# Autodesk Inventor assembly: ForearmActuatorBody
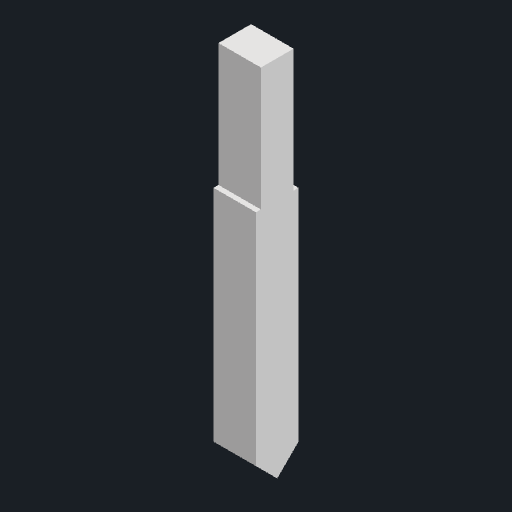
[picture p0: Inventor's stored thumbnail of the model, 512x512]
Saved by Autodesk Inventor 2023 (Build 270158000, 158)
## iProperties
Created: 2023-03-25
Part Number: ForearmActuatorBody
Document SubType Name: Assembly
Designer: Val
Author: Val
## Documents named in this file (3)
- C:\Users\valer\Desktop\str1ker\cad\external\ForearmActuator\ForearmActuatorBody.iam
- C:\Users\valer\Desktop\str1ker\cad\external\ForearmActuator\ForearmActuatorBody.ipt
- C:\Users\valer\Desktop\str1ker\cad\external\ForearmActuator\ForearmActuatorBodyBoundingBoxReal.ipt
## Components (2 placed, 2 different names)
1. ForearmActuatorBody:1 — Angle:1, Angle:2, Mate:1
2. ForearmActuatorBodyBoundingBoxReal:1 — Flush:1
## Relationships (4: Angle 2, Mate 1, Flush 1)
- Angle:1 (180 deg): ForearmActuatorBody:1
- Angle:2 (180 deg): ForearmActuatorBody:1
- Mate:1: ForearmActuatorBody:1
- Flush:1: ForearmActuatorBodyBoundingBoxReal:1
